# Autodesk Inventor assembly: SHELL INTERFACE 1
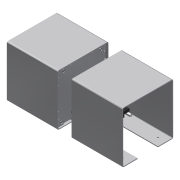
[picture p0: Inventor's stored thumbnail of the model, 180x180]
Saved by Autodesk Inventor 2018 (Build 220112000, 112)
## iProperties
Created: 2018-12-18
Part Number: SHELL INTERFACE 1
Document SubType Name: Assembly
Designer: R.P.SMITH
Mass: 429.443 g
Surface Area: 2538.74 cm^2
Volume: 183.779 cm^3
Density: 2.33674 g/cm^3
Author: R.P.SMITH
## Documents named in this file (12)
- D:\Documents\College\Semesters\4 - Fall\Senior Project 2\CADD Files\INTERFACE 1.iam
- D:\Documents\College\Semesters\4 - Fall\Senior Project 2\CADD Files\Custom Parts\SEGMENT SHELL.ipt
- D:\Documents\College\Semesters\4 - Fall\Senior Project 2\CADD Files\PC104 ISA BOARD.iam
- D:\Documents\College\Semesters\4 - Fall\Senior Project 2\CADD Files\McMaster\91772A106_18-8 SS PAN HEAD PHILLIPS MACHINE SCREW.ipt
- D:\Documents\College\Semesters\4 - Fall\Senior Project 2\CADD Files\McMaster\93505A925_ALUM MALE-FEM THRDED HEX STANDOFF.ipt
- D:\Documents\College\Semesters\4 - Fall\Senior Project 2\CADD Files\Mouser\SSQ-120-23-G-D.ipt
- D:\Documents\College\Semesters\4 - Fall\Senior Project 2\CADD Files\Custom Parts\END MOUNT PC104 TOP INTERFACE 1.iam
- D:\Documents\College\Semesters\4 - Fall\Senior Project 2\CADD Files\Custom Parts\END MOUNT PC104 BOTTOM INTERFACE 1.ipt
- D:\Documents\College\Semesters\4 - Fall\Senior Project 2\CADD Files\McMaster\92510A692_ALUM UNTHRD SPACER.ipt
- D:\Documents\College\Semesters\4 - Fall\Senior Project 2\CADD Files\McMaster\91772A112_18-8 SS PAN HEAD PHILLIPS MACHINE SCREW.ipt
- D:\Documents\College\Semesters\4 - Fall\Senior Project 2\CADD Files\McMaster\91780A534_ALUM FEM THRDED HEX STANDOFF.ipt
- D:\Documents\College\Semesters\4 - Fall\Senior Project 2\CADD Files\PC104 ISA CUT INTERFACE 1.iam
## Components (27 placed, 11 different names)
1. SEGMENT SHELL:1 — Flush:2, Flush:3, Mate:7, Mate:8, Flush:4
2. END MOUNT PC104 TOP INTERFACE 1:1 [sub-assembly] — Insert:10, Insert:11, Insert:12, Insert:13, Insert:14, Insert:15, Insert:16, Insert:17, Mate:7, Mate:8, Flush:4
3. PC104 ISA BOARD:1 [sub-assembly] — Mate:5, Mate:6, Insert:9, Insert:18, Mate:9
4. 91772A106_18-8 SS PAN HEAD PHILLIPS MACHINE SCREW:1 — Insert:14
5. 91772A106_18-8 SS PAN HEAD PHILLIPS MACHINE SCREW:2 — Insert:15
6. 91772A106_18-8 SS PAN HEAD PHILLIPS MACHINE SCREW:3 — Insert:16
7. 91772A106_18-8 SS PAN HEAD PHILLIPS MACHINE SCREW:4 — Insert:10
8. 93505A925_ALUM MALE-FEM THRDED HEX STANDOFF:1 — Insert:12
9. 93505A925_ALUM MALE-FEM THRDED HEX STANDOFF:2 — Insert:11
10. 93505A925_ALUM MALE-FEM THRDED HEX STANDOFF:3 — Insert:17, Insert:18
11. 93505A925_ALUM MALE-FEM THRDED HEX STANDOFF:4 — Insert:9, Insert:13
12. SSQ-120-23-G-D:1 — Mate:5, Mate:6, Mate:9
13. SEGMENT SHELL:2 — Flush:2, Flush:3, Mate:10, Mate:11, Flush:5
14. END MOUNT PC104 BOTTOM INTERFACE 1:1 — Mate:10, Mate:11, Mate:12, Mate:13, Insert:20, Insert:21, Insert:22, Insert:23, Insert:24, Insert:25, Insert:26, Insert:27, Flush:5
15. PC104 ISA CUT INTERFACE 1:1 [sub-assembly] — Mate:12, Mate:13, Insert:19, Insert:28, Insert:29, Insert:30, Insert:31
16. 92510A692_ALUM UNTHRD SPACER:1 — Insert:19, Insert:20
17. 92510A692_ALUM UNTHRD SPACER:2 — Insert:23
18. 92510A692_ALUM UNTHRD SPACER:3 — Insert:21
19. 92510A692_ALUM UNTHRD SPACER:4 — Insert:22
20. 91772A112_18-8 SS PAN HEAD PHILLIPS MACHINE SCREW:1 — Insert:24
21. 91772A112_18-8 SS PAN HEAD PHILLIPS MACHINE SCREW:2 — Insert:25
22. 91772A112_18-8 SS PAN HEAD PHILLIPS MACHINE SCREW:3 — Insert:26
23. 91772A112_18-8 SS PAN HEAD PHILLIPS MACHINE SCREW:4 — Insert:27
24. 91780A534_ALUM FEM THRDED HEX STANDOFF:1 — Insert:29
25. 91780A534_ALUM FEM THRDED HEX STANDOFF:2 — Insert:31
26. 91780A534_ALUM FEM THRDED HEX STANDOFF:3 — Insert:30
27. 91780A534_ALUM FEM THRDED HEX STANDOFF:4 — Insert:28
## Relationships (36: Insert 23, Mate 9, Flush 4)
- Mate:5: PC104 ISA BOARD:1 ↔ SSQ-120-23-G-D:1
- Mate:6: PC104 ISA BOARD:1 ↔ SSQ-120-23-G-D:1
- Insert:9: PC104 ISA BOARD:1 ↔ 93505A925_ALUM MALE-FEM THRDED HEX STANDOFF:4
- Flush:2: SEGMENT SHELL:1 ↔ SEGMENT SHELL:2
- Flush:3: SEGMENT SHELL:1 ↔ SEGMENT SHELL:2
- Insert:10: END MOUNT PC104 TOP INTERFACE 1:1 ↔ 91772A106_18-8 SS PAN HEAD PHILLIPS MACHINE SCREW:4
- Insert:11: END MOUNT PC104 TOP INTERFACE 1:1 ↔ 93505A925_ALUM MALE-FEM THRDED HEX STANDOFF:2
- Insert:12: END MOUNT PC104 TOP INTERFACE 1:1 ↔ 93505A925_ALUM MALE-FEM THRDED HEX STANDOFF:1
- Insert:13: END MOUNT PC104 TOP INTERFACE 1:1 ↔ 93505A925_ALUM MALE-FEM THRDED HEX STANDOFF:4
- Insert:14: END MOUNT PC104 TOP INTERFACE 1:1 ↔ 91772A106_18-8 SS PAN HEAD PHILLIPS MACHINE SCREW:1
- Insert:15: END MOUNT PC104 TOP INTERFACE 1:1 ↔ 91772A106_18-8 SS PAN HEAD PHILLIPS MACHINE SCREW:2
- Insert:16: END MOUNT PC104 TOP INTERFACE 1:1 ↔ 91772A106_18-8 SS PAN HEAD PHILLIPS MACHINE SCREW:3
- Insert:17: END MOUNT PC104 TOP INTERFACE 1:1 ↔ 93505A925_ALUM MALE-FEM THRDED HEX STANDOFF:3
- Mate:7 (0.25 mm): SEGMENT SHELL:1 ↔ END MOUNT PC104 TOP INTERFACE 1:1
- Mate:8 (0.25 mm): SEGMENT SHELL:1 ↔ END MOUNT PC104 TOP INTERFACE 1:1
- Insert:18: PC104 ISA BOARD:1 ↔ 93505A925_ALUM MALE-FEM THRDED HEX STANDOFF:3
- Flush:4 (2.5 mm): SEGMENT SHELL:1 ↔ END MOUNT PC104 TOP INTERFACE 1:1
- Mate:9 (4 mm): PC104 ISA BOARD:1 ↔ SSQ-120-23-G-D:1
- Mate:10 (0.25 mm): SEGMENT SHELL:2 ↔ END MOUNT PC104 BOTTOM INTERFACE 1:1
- Mate:11 (0.25 mm): SEGMENT SHELL:2 ↔ END MOUNT PC104 BOTTOM INTERFACE 1:1
- Mate:12: END MOUNT PC104 BOTTOM INTERFACE 1:1 ↔ PC104 ISA CUT INTERFACE 1:1
- Mate:13: END MOUNT PC104 BOTTOM INTERFACE 1:1 ↔ PC104 ISA CUT INTERFACE 1:1
- Insert:19: PC104 ISA CUT INTERFACE 1:1 ↔ 92510A692_ALUM UNTHRD SPACER:1
- Insert:20: END MOUNT PC104 BOTTOM INTERFACE 1:1 ↔ 92510A692_ALUM UNTHRD SPACER:1
- Insert:21: END MOUNT PC104 BOTTOM INTERFACE 1:1 ↔ 92510A692_ALUM UNTHRD SPACER:3
- Insert:22: END MOUNT PC104 BOTTOM INTERFACE 1:1 ↔ 92510A692_ALUM UNTHRD SPACER:4
- Insert:23: END MOUNT PC104 BOTTOM INTERFACE 1:1 ↔ 92510A692_ALUM UNTHRD SPACER:2
- Insert:24: END MOUNT PC104 BOTTOM INTERFACE 1:1 ↔ 91772A112_18-8 SS PAN HEAD PHILLIPS MACHINE SCREW:1
- Insert:25: END MOUNT PC104 BOTTOM INTERFACE 1:1 ↔ 91772A112_18-8 SS PAN HEAD PHILLIPS MACHINE SCREW:2
- Insert:26: END MOUNT PC104 BOTTOM INTERFACE 1:1 ↔ 91772A112_18-8 SS PAN HEAD PHILLIPS MACHINE SCREW:3
- Insert:27: END MOUNT PC104 BOTTOM INTERFACE 1:1 ↔ 91772A112_18-8 SS PAN HEAD PHILLIPS MACHINE SCREW:4
- Insert:28: PC104 ISA CUT INTERFACE 1:1 ↔ 91780A534_ALUM FEM THRDED HEX STANDOFF:4
- Insert:29: PC104 ISA CUT INTERFACE 1:1 ↔ 91780A534_ALUM FEM THRDED HEX STANDOFF:1
- Insert:30: PC104 ISA CUT INTERFACE 1:1 ↔ 91780A534_ALUM FEM THRDED HEX STANDOFF:3
- Insert:31: PC104 ISA CUT INTERFACE 1:1 ↔ 91780A534_ALUM FEM THRDED HEX STANDOFF:2
- Flush:5 (2 mm): SEGMENT SHELL:2 ↔ END MOUNT PC104 BOTTOM INTERFACE 1:1
